# Autodesk Inventor assembly: assembly
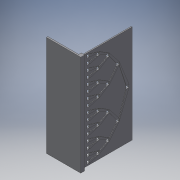
[picture p0: Inventor's stored thumbnail of the model, 180x180]
Saved by Autodesk Inventor 2018.2 (Build 222227000, 227)
## iProperties
Created: 2018-01-31
Part Number: assembly
Document SubType Name: Assembly
Designer: wharr
Author: wharr
## Documents named in this file (3)
- C:\MEGA\NCSSM\CS434 Data Structures I\neopixel tree\parts\assembly.iam
- C:\MEGA\NCSSM\CS434 Data Structures I\neopixel tree\parts\base.ipt
- C:\MEGA\NCSSM\CS434 Data Structures I\neopixel tree\parts\front plate.ipt
## Components (2 placed, 2 different names)
1. base:1 — Mate:1, Mate:2, Mate:3
2. front plate:1 — Mate:1, Mate:2, Mate:3
## Relationships (3: Mate 3)
- Mate:1: base:1 ↔ front plate:1
- Mate:2: base:1 ↔ front plate:1
- Mate:3: base:1 ↔ front plate:1
